# Autodesk Inventor assembly: Race Inner nema 23
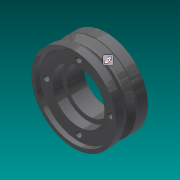
[picture p0: Inventor's stored thumbnail of the model, 180x180]
Saved by Autodesk Inventor 2020.3 (Build 243373000, 373)
## iProperties
Created: 2020-05-22
Part Number: Race Inner nema 23
Document SubType Name: Assembly
Designer: Administrator
Title: Race Inner
Author: Administrator
## Documents named in this file (3)
- C:\Users\Svend\OneDrive\Documents\GitHub\BeerMinder\3D-model\bearings\slewbearing\Race Inner nema 23.iam
- C:\Users\Svend\OneDrive\Documents\GitHub\BeerMinder\3D-model\bearings\slewbearing\slewbearing nema23\Race Inner Bottom v2.ipt
- C:\Users\Svend\OneDrive\Documents\GitHub\BeerMinder\3D-model\bearings\slewbearing\slewbearing nema23\Race Inner Top v2.ipt
## Components (2 placed, 2 different names)
1. Race Inner Bottom v2:1 — Mate:1, Mate:4
2. Race Inner Top v2:1 — Mate:1, Mate:4
## Relationships (3: Mate 3)
- Mate:1: Race Inner Bottom v2:1 ↔ Race Inner Top v2:1
- [Mate]: Race Inner Bottom v2:1 ↔ Race Inner Top v2:1
- Mate:4: Race Inner Bottom v2:1 ↔ Race Inner Top v2:1
